# Autodesk Inventor assembly: assembly
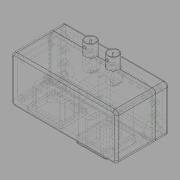
[picture p0: Inventor's stored thumbnail of the model, 180x180]
Saved by Autodesk Inventor 2013 (Build 170138000, 138)
## iProperties
Created: 2014-06-08
Part Number: assembly
Document SubType Name: Assembly
Designer: Brad
Author: Brad
## Documents named in this file (8)
- C:\Users\Brad\Documents\GitHub\wAveC\case\assembly.iam
- C:\Users\Brad\Documents\GitHub\wAveC\case\case_bottom.ipt
- C:\Users\Brad\Documents\GitHub\wAveC\case\pcb.ipt
- C:\Users\Brad\Documents\GitHub\wAveC\case\0731000105.ipt
- C:\Users\Brad\Documents\GitHub\wAveC\case\cr8348-1000.ipt
- C:\Users\Brad\Documents\GitHub\wAveC\case\case_top.ipt
- C:\Users\Brad\Documents\GitHub\wAveC\case\701W-X202.ipt
- C:\Users\Brad\Documents\GitHub\wAveC\case\739W-X203.ipt
## Components (8 placed, 7 different names)
1. case_bottom:1 — Insert:1, Insert:2, Insert:9, Insert:10, Mate:4
2. pcb:1 — Insert:1, Insert:2, Mate:1, Insert:3, Insert:4, Mate:2, Insert:5, Insert:6, Mate:3, Insert:7, Insert:8
3. 0731000105:1 — Mate:1, Insert:3, Insert:4
4. 0731000105:2 — Mate:2, Insert:5, Insert:6
5. cr8348-1000:1 — Mate:3, Insert:7, Insert:8
6. case_top:1 — Insert:9, Insert:10, Mate:4, Mate:5, Mate:6, Mate:7, Mate:8, Mate:9, Mate:10
7. 701W-X202:1 — Mate:8, Mate:9, Mate:10
8. 739W-X203:1 — Mate:5, Mate:6, Mate:7
## Relationships (20: Insert 10, Mate 10)
- Insert:1: case_bottom:1 ↔ pcb:1
- Insert:2: case_bottom:1 ↔ pcb:1
- Mate:1: pcb:1 ↔ 0731000105:1
- Insert:3: pcb:1 ↔ 0731000105:1
- Insert:4: pcb:1 ↔ 0731000105:1
- Mate:2: pcb:1 ↔ 0731000105:2
- Insert:5: pcb:1 ↔ 0731000105:2
- Insert:6: pcb:1 ↔ 0731000105:2
- Mate:3: pcb:1 ↔ cr8348-1000:1
- Insert:7: pcb:1 ↔ cr8348-1000:1
- Insert:8: pcb:1 ↔ cr8348-1000:1
- Insert:9: case_bottom:1 ↔ case_top:1
- Insert:10: case_bottom:1 ↔ case_top:1
- Mate:4: case_bottom:1 ↔ case_top:1
- Mate:5: case_top:1 ↔ 739W-X203:1
- Mate:6: case_top:1 ↔ 739W-X203:1
- Mate:7: case_top:1 ↔ 739W-X203:1
- Mate:8: case_top:1 ↔ 701W-X202:1
- Mate:9: case_top:1 ↔ 701W-X202:1
- Mate:10: case_top:1 ↔ 701W-X202:1
